# Autodesk Inventor assembly: Shock Strut
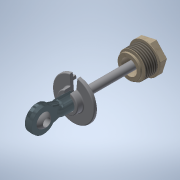
[picture p0: Inventor's stored thumbnail of the model, 180x180]
Saved by Autodesk Inventor 2022.3 (Build 263350000, 350)
## iProperties
Created: 2019-12-01
Part Number: Shock Strut
Document SubType Name: Assembly
Designer: Jopa
Author: Jopa
## Documents named in this file (6)
- D:\Luis\Desktop\ESPOL\9 semestre\Itinerario\PIEZAS\PX9200-18_Front-Rear_Shock_Absorber\Shock Strut\Shock Strut.iam
- D:\Luis\Desktop\ESPOL\9 semestre\Itinerario\PIEZAS\PX9200-18_Front-Rear_Shock_Absorber\Shock Strut\Shock Shaft.ipt
- D:\Luis\Desktop\ESPOL\9 semestre\Itinerario\PIEZAS\PX9200-18_Front-Rear_Shock_Absorber\Shock Body\Shock Cartridge\Shock Cartridge.ipt
- D:\Luis\Desktop\ESPOL\9 semestre\Itinerario\PIEZAS\PX9200-18_Front-Rear_Shock_Absorber\Shock Strut\E-Clip.ipt
- D:\Luis\Desktop\ESPOL\9 semestre\Itinerario\PIEZAS\PX9200-18_Front-Rear_Shock_Absorber\Shock Strut\Ball End.iam
- D:\Luis\Desktop\ESPOL\9 semestre\Itinerario\PIEZAS\PX9200-18_Front-Rear_Shock_Absorber\Shock Strut\Spring Cup.ipt
## Components (6 placed, 5 different names)
1. Shock Shaft:1 — Mate:1, Flush:1, Mate:6, Mate:7, Mate:9
2. Shock Cartridge:1 — Mate:1, Mate:2, Mate:3, Mate:4, Mate:5, Flush:1
3. E-Clip:1 — Mate:4, Mate:5
4. E-Clip:2 — Mate:2, Mate:3
5. Ball End:1 [sub-assembly] — Mate:6, Mate:7, Mate:8
6. Spring Cup:1 — Mate:8, Mate:9
## Relationships (10: Mate 9, Flush 1)
- Mate:1: Shock Shaft:1 ↔ Shock Cartridge:1
- Mate:2: Shock Cartridge:1 ↔ E-Clip:2
- Mate:3: Shock Cartridge:1 ↔ E-Clip:2
- Mate:4: Shock Cartridge:1 ↔ E-Clip:1
- Mate:5: Shock Cartridge:1 ↔ E-Clip:1
- Flush:1: Shock Shaft:1 ↔ Shock Cartridge:1
- Mate:6: Shock Shaft:1 ↔ Ball End:1
- Mate:7: Shock Shaft:1 ↔ Ball End:1
- Mate:8: Ball End:1 ↔ Spring Cup:1
- Mate:9: Shock Shaft:1 ↔ Spring Cup:1
